# Autodesk Inventor assembly: Drive Outside Bracket
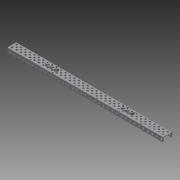
[picture p0: Inventor's stored thumbnail of the model, 180x180]
Saved by Autodesk Inventor 2015 (Build 190159000, 159)
## iProperties
Created: 2016-09-22
Part Number: Drive Outside Bracket
Document SubType Name: Assembly
Designer: Leo
Author: Leo
## Documents named in this file (4)
- C:\Users\Leo\Google Drive\StarStuckProject\Starstruck\Prototypes\Drive Inside Bracket.iam
- C:\Users\Leo\Google Drive\StarStuckProject\Starstruck\Imported Components\C-Channel 1x2x1x35\C-Channel 1x2x1x35.ipt
- C:\Users\Leo\Google Drive\StarStuckProject\Starstruck\Imported Components\Flat Bearing\Flat Bearing.ipt
- C:\Users\Leo\Google Drive\StarStuckProject\Starstruck\Imported Components\Small Screw .50In\Small Screw .50In.ipt
## Components (7 placed, 3 different names)
1. C-Channel 1x2x1x35:1 — Mate:1, Mate:2, Mate:3, Mate:4, Mate:5, Mate:6
2. Flat Bearing:1 — Mate:1, Insert:3, Insert:4
3. Flat Bearing:2 — Mate:2, Insert:1, Insert:2
4. Small Screw .50In:1 — Mate:5, Insert:3
5. Small Screw .50In:2 — Mate:6, Insert:2
6. Small Screw .50In:3 — Mate:4, Insert:4
7. Small Screw .50In:4 — Mate:3, Insert:1
## Relationships (10: Mate 6, Insert 4)
- Mate:1: C-Channel 1x2x1x35:1 ↔ Flat Bearing:1
- Mate:2: C-Channel 1x2x1x35:1 ↔ Flat Bearing:2
- Mate:3: C-Channel 1x2x1x35:1 ↔ Small Screw .50In:4
- Mate:4: C-Channel 1x2x1x35:1 ↔ Small Screw .50In:3
- Mate:5: C-Channel 1x2x1x35:1 ↔ Small Screw .50In:1
- Mate:6: C-Channel 1x2x1x35:1 ↔ Small Screw .50In:2
- Insert:1 (1.1684 mm): Flat Bearing:2 ↔ Small Screw .50In:4
- Insert:2 (1.1684 mm): Flat Bearing:2 ↔ Small Screw .50In:2
- Insert:3 (1.1684 mm): Flat Bearing:1 ↔ Small Screw .50In:1
- Insert:4 (1.1684 mm): Flat Bearing:1 ↔ Small Screw .50In:3
